# Autodesk Inventor assembly: CzujnikUltraDziekowy
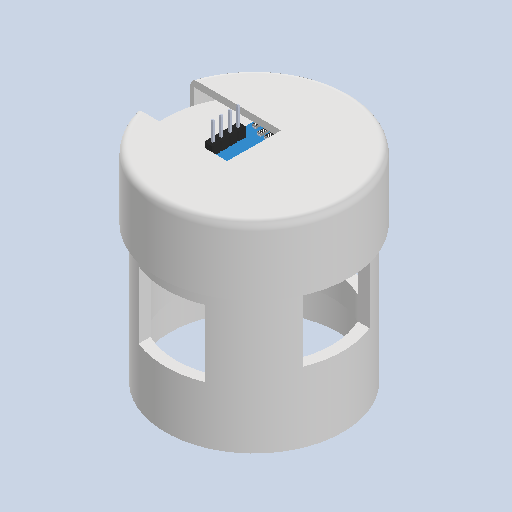
[picture p0: Inventor's stored thumbnail of the model, 512x512]
Saved by Autodesk Inventor 2024.3 (Build 283343000, 343)
## iProperties
Created: 2024-12-26
Part Number: CzujnikUltraDziekowy
Document SubType Name: Assembly
Designer: adamn
Author: adamn
## Documents named in this file (4)
- C:\Users\adamn\Desktop\ProjektSTM\CzujnikUltraDziekowy.iam
- C:\Users\adamn\Desktop\ProjektSTM\ObudowaCzujnika.ipt
- C:\Users\adamn\Desktop\ProjektSTM\ultrasonic-sensor-hc-sr04-3.snapshot.1\HC-SR04\HC-SR04\HC-SR04.iam
- C:\Users\adamn\Desktop\ProjektSTM\PokrywaCzujnika.ipt
## Components (3 placed, 3 different names)
1. ObudowaCzujnika:1 — Wstawiające:1, Wstawiające:2, Wstawiające:3
2. HC-SR04:1 [sub-assembly] — Wstawiające:1, Wstawiające:2
3. PokrywaCzujnika:1 — Wstawiające:3
## Relationships (3: Insert 3)
- Wstawiające:1 [Insert]: ObudowaCzujnika:1 ↔ HC-SR04:1
- Wstawiające:2 [Insert]: ObudowaCzujnika:1 ↔ HC-SR04:1
- Wstawiające:3 [Insert] (4 mm): ObudowaCzujnika:1 ↔ PokrywaCzujnika:1
